# Autodesk Inventor assembly: Pok Mk3
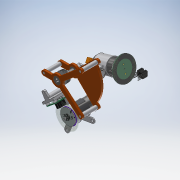
[picture p0: Inventor's stored thumbnail of the model, 180x180]
Saved by Autodesk Inventor 2018.2 (Build 222227000, 227)
## iProperties
Created: 2018-02-12
Part Number: Pok Mk3
Document SubType Name: Assembly
Designer: Moochster
Author: Moochster
## Documents named in this file (23)
- C:\Users\Moochster\OneDrive\Documents\2018 UBC\ELEC 391\Controller\CAD\Pok Mk3.iam
- C:\Users\Moochster\OneDrive\Documents\2018 UBC\ELEC 391\Controller\CAD\Rod 3-8in.ipt
- C:\Users\Moochster\OneDrive\Documents\2018 UBC\ELEC 391\Controller\CAD\R1038_ZZ_W Bearing.ipt
- C:\Users\Moochster\OneDrive\Documents\2018 UBC\ELEC 391\Controller\CAD\Yaw Platform Top.ipt
- C:\Users\Moochster\OneDrive\Documents\2018 UBC\ELEC 391\Controller\CAD\Pok Header Mount.ipt
- C:\Users\Moochster\OneDrive\Documents\2018 UBC\ELEC 391\Controller\CAD\JD5B-2655W-R.ipt
- C:\Users\Moochster\OneDrive\Documents\2018 UBC\ELEC 391\Controller\CAD\Pok Default Pitch Motor Mount.ipt
- C:\Users\Moochster\OneDrive\Documents\2018 UBC\ELEC 391\Controller\CAD\Laser Mount.ipt
- C:\Users\Moochster\Documents\Inventor\Content Center Files\R2018\en-US\AS 1110\AS 1110 - M3 x 20.ipt
- C:\Users\Moochster\Documents\Inventor\Content Center Files\R2018\en-US\AS 1112 (2)\AS 1112 - M3  Type 5.ipt
- C:\Users\Moochster\Documents\Inventor\Content Center Files\R2018\en-US\CNS 5050\CNS 5050 - A - 3.2 8.ipt
- C:\Users\Moochster\Documents\Inventor\Content Center Files\R2018\en-US\ANSI B18.3.1M(1)\ANSI B18.3.1M - M1.6x0.35 x 3(2).ipt
- C:\Users\Moochster\OneDrive\Documents\2018 UBC\ELEC 391\Controller\CAD\Pok Mk3 Base.ipt
- C:\Users\Moochster\OneDrive\Documents\2018 UBC\ELEC 391\Controller\CAD\Pok Mk3 Support.ipt
- C:\Users\Moochster\OneDrive\Documents\2018 UBC\ELEC 391\Controller\CAD\Encoder Wheel (G16).ipt
- C:\Users\Moochster\OneDrive\Documents\2018 UBC\ELEC 391\Controller\CAD\Shaft Encoder Adapter.ipt
- C:\Users\Moochster\OneDrive\Documents\2018 UBC\ELEC 391\Controller\CAD\GP1A52HRJ00F (Large slot detector).ipt
- C:\Users\Moochster\OneDrive\Documents\2018 UBC\ELEC 391\Controller\CAD\GT2 Gear Pinion.ipt
- C:\Users\Moochster\OneDrive\Documents\2018 UBC\ELEC 391\Controller\CAD\GT2 Gear Big.ipt
- C:\Users\Moochster\OneDrive\Documents\2018 UBC\ELEC 391\Controller\CAD\Pok Mk3 Yaw Motor Support.ipt
- C:\Users\Moochster\OneDrive\Documents\2018 UBC\ELEC 391\Controller\CAD\Large Encoder PCB.ipt
- C:\Users\Moochster\OneDrive\Documents\2018 UBC\ELEC 391\Controller\CAD\Nylon M3 4mm Spacer.ipt
- C:\Users\Moochster\OneDrive\Documents\2018 UBC\ELEC 391\Controller\CAD\Pok Mk3 Yaw Motor Mount Mk2.ipt
## Components (40 placed, 22 different names)
1. Rod 3-8in:1 — Mate:1, Mate:2, Flush:1, Mate:10, Mate:23, Mate:24, Flush:6, Mate:42
2. R1038_ZZ_W Bearing:1 — Mate:1, Flush:1
3. R1038_ZZ_W Bearing:2 — Mate:2, Mate:5, Flush:2
4. Yaw Platform Top:1 — Mate:5, Flush:2, Mate:11, Angle:1
5. Pok Header Mount:1 — Mate:10, Mate:11, Mate:12, Flush:4, Mate:19, Mate:20, Mate:21
6. R1038_ZZ_W Bearing:3 — Mate:12, Flush:4
7. JD5B-2655W-R:1 — Mate:17, Mate:18, Mate:22, Flush:5, Angle:2, Tangent:1, Tangent:2, Mate:34, Mate:38
8. Laser Mount:1 — Mate:17, Mate:18
9. Pok Default Pitch Motor Mount:1 — Mate:19, Mate:20, Mate:21, Mate:22, Flush:5, Mate:25, Insert:1, Insert:3, Insert:5, Insert:7, Angle:2, Mate:26, Mate:27
10. AS 1110 - Metric M3 x 20:1 — Mate:25, Insert:2
11. AS 1110 - Metric M3 x 20:2 — Insert:6
12. CNS 5050 A - 3.2:4 — Insert:7, Insert:8
13. CNS 5050 A - 3.2:2 — Insert:5, Insert:6
14. CNS 5050 A - 3.2:3 — Insert:3, Insert:4
15. CNS 5050 A - 3.2:1 — Insert:1, Insert:2
16. AS 1112 (2) - Metric M3  Type 5:1 — Insert:8
17. AS 1112 (2) - Metric M3  Type 5:2 — Insert:4
18. Broached Socket Head Cap Screw - Metric M1.6x0.35 x 3:1 — Mate:26, Tangent:1
19. Broached Socket Head Cap Screw - Metric M1.6x0.35 x 3:2 — Mate:27, Tangent:2
20. Pok Mk3 Base:1 — Flush:6, Mate:28, Flush:7, Mate:29, Flush:8, Mate:30, Flush:9, Angle:3, Flush:17
21. Pok Mk3 Support:1 — Mate:28, Flush:7
22. Pok Mk3 Support:2 — Mate:30, Flush:9
23. Pok Mk3 Support:3 — Mate:29, Flush:8
24. JD5B-2655W-R:2 — Mate:32, Mate:41, Angle:3, Mate:44, Mate:53, Mate:55
25. Encoder Wheel (G16):1 — Mate:32, Mate:43, Mate:44
26. Encoder Wheel (G16):2 — Mate:35, Mate:36, Mate:37
27. Shaft Encoder Adapter:1 — Mate:34, Mate:35, Mate:36, Mate:37, Mate:38
28. GP1A52HRJ00F (Large slot detector):1 — Mate:39, Mate:40
29. GP1A52HRJ00F (Large slot detector):2 — Mate:39, Mate:40
30. GP1A52HRJ00F (Large slot detector):3 — Mate:50, Flush:13, Flush:14, Mate:51, Flush:15
31. GP1A52HRJ00F (Large slot detector):4 — Mate:50, Flush:13, Flush:14, Flush:16
32. GT2 Gear Pinion:1 — Mate:41, Mate:43, Flush:10
33. GT2 Gear Big:1 — Mate:42, Flush:10
34. Pok Mk3 Yaw Motor Support:4 — Mate:48, Mate:49, Mate:52, Insert:9, Insert:10, Insert:11, Insert:12, Mate:54, Angle:4, Insert:13, Flush:17
35. Large Encoder PCB:1 — Mate:48, Mate:49, Mate:51, Flush:15, Flush:16, Mate:52
36. Nylon M3 4mm Spacer:1 — Insert:11
37. Nylon M3 4mm Spacer:2 — Insert:9
38. Nylon M3 4mm Spacer:3 — Insert:10
39. Nylon M3 4mm Spacer:4 — Insert:12
40. Pok Mk3 Yaw Motor Mount Mk2:1 — Mate:53, Mate:54, Angle:4, Insert:13, Mate:55
## Relationships (73: Mate 40, Flush 14, Insert 13, Angle 4, Tangent 2)
- Mate:1: Rod 3-8in:1 ↔ R1038_ZZ_W Bearing:1
- Mate:2: Rod 3-8in:1 ↔ R1038_ZZ_W Bearing:2
- Flush:1: Rod 3-8in:1 ↔ R1038_ZZ_W Bearing:1
- Mate:5: R1038_ZZ_W Bearing:2 ↔ Yaw Platform Top:1
- Flush:2: R1038_ZZ_W Bearing:2 ↔ Yaw Platform Top:1
- Mate:10: Rod 3-8in:1 ↔ Pok Header Mount:1
- Mate:11 (0.2 mm): Yaw Platform Top:1 ↔ Pok Header Mount:1
- Mate:12: Pok Header Mount:1 ↔ R1038_ZZ_W Bearing:3
- Flush:4 (1 mm): Pok Header Mount:1 ↔ R1038_ZZ_W Bearing:3
- Mate:17: JD5B-2655W-R:1 ↔ Laser Mount:1
- Mate:18 (1 mm): JD5B-2655W-R:1 ↔ Laser Mount:1
- Mate:19: Pok Header Mount:1 ↔ Pok Default Pitch Motor Mount:1
- Mate:20: Pok Header Mount:1 ↔ Pok Default Pitch Motor Mount:1
- Mate:21 (0.1 mm): Pok Header Mount:1 ↔ Pok Default Pitch Motor Mount:1
- Mate:22: JD5B-2655W-R:1 ↔ Pok Default Pitch Motor Mount:1
- Mate:23: Rod 3-8in:1
- Mate:24: Rod 3-8in:1
- Angle:1 (0 deg): Yaw Platform Top:1
- Flush:5 (-10 mm): JD5B-2655W-R:1 ↔ Pok Default Pitch Motor Mount:1
- Mate:25: Pok Default Pitch Motor Mount:1 ↔ AS 1110 - Metric M3 x 20:1
- Insert:1: Pok Default Pitch Motor Mount:1 ↔ CNS 5050 A - 3.2:1
- Insert:2: AS 1110 - Metric M3 x 20:1 ↔ CNS 5050 A - 3.2:1
- Insert:3: Pok Default Pitch Motor Mount:1 ↔ CNS 5050 A - 3.2:3
- Insert:4: CNS 5050 A - 3.2:3 ↔ AS 1112 (2) - Metric M3  Type 5:2
- Insert:5: Pok Default Pitch Motor Mount:1 ↔ CNS 5050 A - 3.2:2
- Insert:6: AS 1110 - Metric M3 x 20:2 ↔ CNS 5050 A - 3.2:2
- Insert:7: Pok Default Pitch Motor Mount:1 ↔ CNS 5050 A - 3.2:4
- Insert:8: CNS 5050 A - 3.2:4 ↔ AS 1112 (2) - Metric M3  Type 5:1
- Angle:2 (180 deg): JD5B-2655W-R:1 ↔ Pok Default Pitch Motor Mount:1
- Mate:26: Pok Default Pitch Motor Mount:1 ↔ Broached Socket Head Cap Screw - Metric M1.6x0.35 x 3:1
- Tangent:1: JD5B-2655W-R:1 ↔ Broached Socket Head Cap Screw - Metric M1.6x0.35 x 3:1
- Mate:27: Pok Default Pitch Motor Mount:1 ↔ Broached Socket Head Cap Screw - Metric M1.6x0.35 x 3:2
- Tangent:2: JD5B-2655W-R:1 ↔ Broached Socket Head Cap Screw - Metric M1.6x0.35 x 3:2
- Flush:6: Rod 3-8in:1 ↔ Pok Mk3 Base:1
- Mate:28: Pok Mk3 Base:1 ↔ Pok Mk3 Support:1
- Flush:7: Pok Mk3 Base:1 ↔ Pok Mk3 Support:1
- Mate:29: Pok Mk3 Base:1 ↔ Pok Mk3 Support:3
- Flush:8: Pok Mk3 Base:1 ↔ Pok Mk3 Support:3
- Mate:30: Pok Mk3 Base:1 ↔ Pok Mk3 Support:2
- Flush:9: Pok Mk3 Base:1 ↔ Pok Mk3 Support:2
- Mate:32: JD5B-2655W-R:2 ↔ Encoder Wheel (G16):1
- Mate:34: JD5B-2655W-R:1 ↔ Shaft Encoder Adapter:1
- Mate:35: Encoder Wheel (G16):2 ↔ Shaft Encoder Adapter:1
- Mate:36: Encoder Wheel (G16):2 ↔ Shaft Encoder Adapter:1
- Mate:37: Encoder Wheel (G16):2 ↔ Shaft Encoder Adapter:1
- Mate:38 (0.25 mm): JD5B-2655W-R:1 ↔ Shaft Encoder Adapter:1
- Mate:39: GP1A52HRJ00F (Large slot detector):1 ↔ GP1A52HRJ00F (Large slot detector):2
- Mate:40: GP1A52HRJ00F (Large slot detector):1 ↔ GP1A52HRJ00F (Large slot detector):2
- Mate:41: JD5B-2655W-R:2 ↔ GT2 Gear Pinion:1
- Angle:3 (0 deg): Pok Mk3 Base:1 ↔ JD5B-2655W-R:2
- Mate:42: Rod 3-8in:1 ↔ GT2 Gear Big:1
- Mate:43: Encoder Wheel (G16):1 ↔ GT2 Gear Pinion:1
- Mate:44 (0.5 mm): JD5B-2655W-R:2 ↔ Encoder Wheel (G16):1
- Flush:10: GT2 Gear Pinion:1 ↔ GT2 Gear Big:1
- Mate:48: Pok Mk3 Yaw Motor Support:4 ↔ Large Encoder PCB:1
- Mate:49: Pok Mk3 Yaw Motor Support:4 ↔ Large Encoder PCB:1
- Mate:50 (0.7 mm): GP1A52HRJ00F (Large slot detector):3 ↔ GP1A52HRJ00F (Large slot detector):4
- Flush:13: GP1A52HRJ00F (Large slot detector):3 ↔ GP1A52HRJ00F (Large slot detector):4
- Flush:14: GP1A52HRJ00F (Large slot detector):3 ↔ GP1A52HRJ00F (Large slot detector):4
- Mate:51 (0.1 mm): GP1A52HRJ00F (Large slot detector):3 ↔ Large Encoder PCB:1
- Flush:15 (2 mm): GP1A52HRJ00F (Large slot detector):3 ↔ Large Encoder PCB:1
- Flush:16 (7 mm): GP1A52HRJ00F (Large slot detector):4 ↔ Large Encoder PCB:1
- Mate:52 (4 mm): Pok Mk3 Yaw Motor Support:4 ↔ Large Encoder PCB:1
- Insert:9: Pok Mk3 Yaw Motor Support:4 ↔ Nylon M3 4mm Spacer:2
- Insert:10: Pok Mk3 Yaw Motor Support:4 ↔ Nylon M3 4mm Spacer:3
- Insert:11: Pok Mk3 Yaw Motor Support:4 ↔ Nylon M3 4mm Spacer:1
- Insert:12: Pok Mk3 Yaw Motor Support:4 ↔ Nylon M3 4mm Spacer:4
- Mate:53: JD5B-2655W-R:2 ↔ Pok Mk3 Yaw Motor Mount Mk2:1
- Mate:54: Pok Mk3 Yaw Motor Support:4 ↔ Pok Mk3 Yaw Motor Mount Mk2:1
- Angle:4 (0 deg): Pok Mk3 Yaw Motor Support:4 ↔ Pok Mk3 Yaw Motor Mount Mk2:1
- Insert:13 (0.1 mm): Pok Mk3 Yaw Motor Support:4 ↔ Pok Mk3 Yaw Motor Mount Mk2:1
- Mate:55: JD5B-2655W-R:2 ↔ Pok Mk3 Yaw Motor Mount Mk2:1
- Flush:17: Pok Mk3 Base:1 ↔ Pok Mk3 Yaw Motor Support:4
